# Autodesk Inventor assembly: ETZ
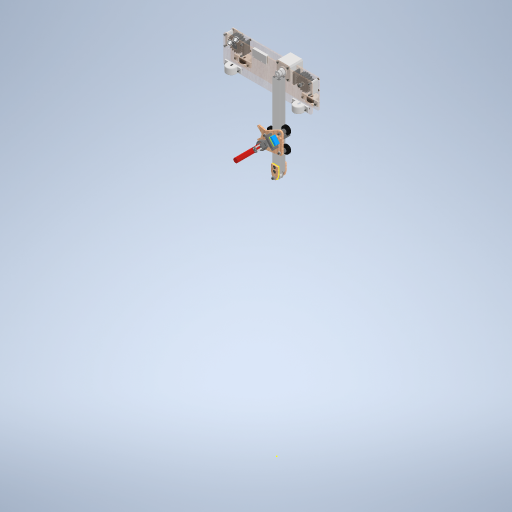
[picture p0: Inventor's stored thumbnail of the model, 512x512]
Saved by Autodesk Inventor 2024 (Build 280153000, 153)
## iProperties
Created: 2026-02-04
Part Number: ETZ
Document SubType Name: Assembly
Designer: SEMEN
Author: SEMEN
## Documents named in this file (4)
- C:\Users\SEMEN\Documents\ETZ2.0\construction\ETZ.iam
- C:\Users\SEMEN\Documents\ETZ2.0\construction\x_axis.iam
- C:\Users\SEMEN\Documents\ETZ2.0\construction\y_axis.iam
- C:\Users\SEMEN\Documents\Inventor\Content Center Files\R2024\en-US\ISO 7046-1 H(1)\ISO 7046-1 - M3 x 8_ - 4.8 - H - ISO.ipt
## Components (6 placed, 3 different names)
1. x_axis:1 [sub-assembly] — Mate:1, Tangent:1, Angle:1, Tangent:2, Mate:2, Mate:3, Mate:4, Mate:5
2. y_axis [sub-assembly] — Mate:1, Tangent:1, Angle:1, Tangent:2
3. ISO 7046-1 H M3 x 8 - 4.8 - H:1 — Mate:2
4. ISO 7046-1 H M3 x 8 - 4.8 - H:2 — Mate:3
5. ISO 7046-1 H M3 x 8 - 4.8 - H:3 — Mate:4
6. ISO 7046-1 H M3 x 8 - 4.8 - H:4 — Mate:5
## Relationships (8: Mate 5, Tangent 2, Angle 1)
- Mate:1: x_axis:1 ↔ y_axis
- Tangent:1 (-2 mm): x_axis:1 ↔ y_axis
- Angle:1 (0 deg): x_axis:1 ↔ y_axis
- Tangent:2 (15 mm): x_axis:1 ↔ y_axis
- Mate:2: x_axis:1 ↔ ISO 7046-1 H M3 x 8 - 4.8 - H:1
- Mate:3: x_axis:1 ↔ ISO 7046-1 H M3 x 8 - 4.8 - H:2
- Mate:4: x_axis:1 ↔ ISO 7046-1 H M3 x 8 - 4.8 - H:3
- Mate:5: x_axis:1 ↔ ISO 7046-1 H M3 x 8 - 4.8 - H:4
